# Autodesk Inventor assembly: Assembly
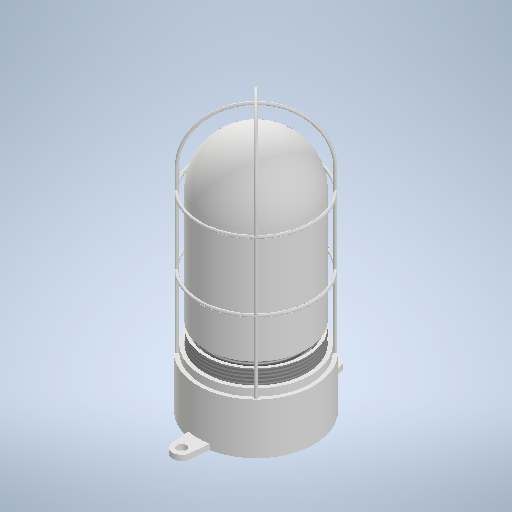
[picture p0: Inventor's stored thumbnail of the model, 512x512]
Saved by Autodesk Inventor 2025.2 (Build 292293000, 293)
## iProperties
Created: 2025-09-04
Part Number: Assembly
Document SubType Name: Assembly
Designer: User
Author: User
## Documents named in this file (3)
- C:\Users\User\Documents\Tagayom Files\revit\mcdonalds-bim\modeling\Assembly.iam
- C:\Users\User\Documents\Tagayom Files\revit\mcdonalds-bim\modeling\base.ipt
- C:\Users\User\Documents\Tagayom Files\revit\mcdonalds-bim\modeling\bulb.ipt
## Components (2 placed, 2 different names)
1. base:1 — Rotational:1
2. bulb:1 — Rotational:1
## Relationships (1: RevoluteJoint 1)
- Rotational:1 [RevoluteJoint] (4.7625 mm): base:1 ↔ bulb:1
